# Autodesk Inventor assembly: Surub M4 saiba piulita 45mm
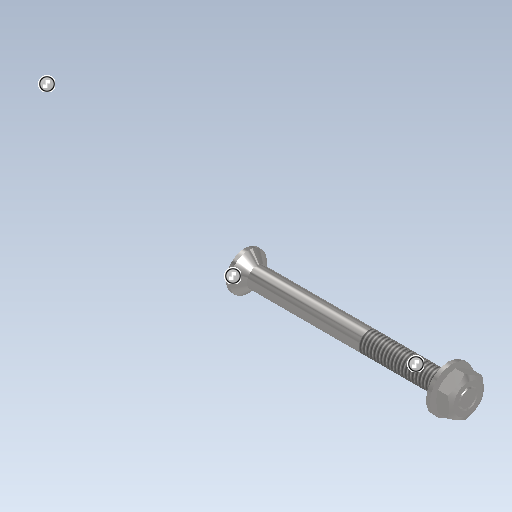
[picture p0: Inventor's stored thumbnail of the model, 512x512]
Saved by Autodesk Inventor 2020 (Build 240168000, 168)
## iProperties
Created: 2020-12-24
Part Number: Surub M4 saiba piulita 45mm
Document SubType Name: Assembly
Designer: Iulian Bors
Author: Iulian Bors
## Documents named in this file (4)
- Z:\I.A.B\Proiecte\0005 I.A.B 3d 2.0 Imprimanta aracet\10 Mecanic\Surub M4 saiba piulita 45mm.iam
- Z:\I.A.B\Proiecte\0005 I.A.B 3d 2.0 Imprimanta aracet\10 Mecanic\0005-10-1039 DIN 7991 - M4  x  45.ipt
- Z:\I.A.B\Proiecte\0005 I.A.B 3d 2.0 Imprimanta aracet\10 Mecanic\0005-10-1014 ISO 4032 - M4 - ISO.ipt
- Z:\I.A.B\Proiecte\0005 I.A.B 3d 2.0 Imprimanta aracet\10 Mecanic\0005-10-1013 ISO 7089 - 4 - 140 HV.ipt
## Components (3 placed, 3 different names)
1. 0005-10-1039 DIN 7991 - M4  x  45.ipt:1 — Insert:1
2. 0005-10-1014 ISO 4032 - M4 - ISO.ipt:2 — Insert:1, Insert:2
3. 0005-10-1013 ISO 7089 - 4 - 140 HV.ipt:3 — Insert:2
## Relationships (2: Insert 2)
- Insert:1: 0005-10-1039 DIN 7991 - M4  x  45.ipt:1 ↔ 0005-10-1014 ISO 4032 - M4 - ISO.ipt:2
- Insert:2: 0005-10-1014 ISO 4032 - M4 - ISO.ipt:2 ↔ 0005-10-1013 ISO 7089 - 4 - 140 HV.ipt:3
